# Autodesk Inventor assembly: Aero_assembly_skid+air
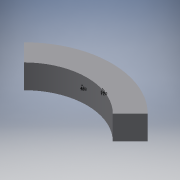
[picture p0: Inventor's stored thumbnail of the model, 180x180]
Saved by Autodesk Inventor 2018.2 (Build 222227000, 227)
## iProperties
Created: 2018-05-17
Part Number: Aero_assembly_skid+air
Material: 一般
Document SubType Name: Assembly
Designer: ku_sk
Author: ku_sk
## Documents named in this file (3)
- D:\ku_sk\ドキュメント\Inventor\Aero\KS-15\Aero_assembly_skid+air.iam
- D:\ku_sk\ドキュメント\Inventor\Aero\KS-15\cradle\base_model\air_skidpad.ipt
- D:\ku_sk\ドキュメント\Inventor\Aero\KS-15\Aero_assembly_skid.iam
## Components (2 placed, 2 different names)
1. air_skidpad:1 — メイト:1, メイト:2, メイト:3, フラッシュ:1
2. Aero_assembly_skid:1 [sub-assembly] — フラッシュ:1, 角度:1, メイト:4
## Relationships (6: Mate 4, Flush 1, Angle 1)
- メイト:1 [Mate]: air_skidpad:1
- メイト:2 [Mate]: air_skidpad:1
- メイト:3 [Mate]: air_skidpad:1
- フラッシュ:1 [Flush] (-30 mm): air_skidpad:1 ↔ Aero_assembly_skid:1
- 角度:1 [Angle] (-2.2 deg): Aero_assembly_skid:1
- メイト:4 [Mate]: Aero_assembly_skid:1
